# Autodesk Inventor assembly: Assembly
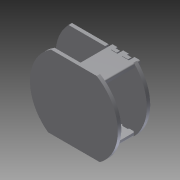
[picture p0: Inventor's stored thumbnail of the model, 180x180]
Saved by Autodesk Inventor 2012 (Build 160160000, 160)
## iProperties
Created: 2013-01-02
Part Number: Assembly
Document SubType Name: Assembly
Designer: asimov
Author: asimov
## Documents named in this file (4)
- C:\Users\asimov\Documents\GitHub\SwarmUSM\Inventor 2012\Assembly.iam
- C:\Users\asimov\Documents\GitHub\SwarmUSM\Inventor 2012\base.ipt
- C:\Users\asimov\Documents\GitHub\SwarmUSM\Inventor 2012\parteA.ipt
- C:\Users\asimov\Documents\GitHub\SwarmUSM\Inventor 2012\superior.ipt
## Components (4 placed, 3 different names)
1. parteA:1 — Mate:1, Mate:3, Mate:4
2. parteA:2 — Mate:2, Mate:5, Mate:6
3. superior:1 — Mate:1, Mate:2
4. base:1 — Mate:3, Mate:4, Mate:5, Mate:6
## Relationships (6: Mate 6)
- Mate:1: parteA:1 ↔ superior:1
- Mate:2: parteA:2 ↔ superior:1
- Mate:3: parteA:1 ↔ base:1
- Mate:4: parteA:1 ↔ base:1
- Mate:5: parteA:2 ↔ base:1
- Mate:6: parteA:2 ↔ base:1
